# Autodesk Inventor assembly: Trunk
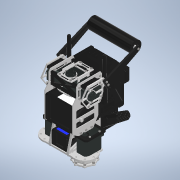
[picture p0: Inventor's stored thumbnail of the model, 180x180]
Saved by Autodesk Inventor 2020.4 (Build 244396000, 396)
## iProperties
Created: 2021-09-10
Part Number: Trunk
Document SubType Name: Assembly
Designer: Masato
Mass: 1663.74 g
Surface Area: 5902.56 cm^2
Volume: 962.647 cm^3
Density: 1.72829 g/cm^3
Author: Masato
## Documents named in this file (38)
- C:\Users\Masato\Documents\Inventor\CIT Brains_Inventor\OpenPlatform_ver3_0\UpperBody\Trunk\Trunk.iam
- C:\Users\Masato\Documents\Inventor\CIT Brains_Inventor\OpenPlatform_ver3_0\UpperBody\Trunk\Trunk_horizontal_frame_02.ipt
- C:\Users\Masato\Documents\Inventor\CIT Brains_Inventor\OpenPlatform_ver3_0\UpperBody\Trunk\Trunk_horizontal_frame_03.ipt
- C:\Users\Masato\Documents\Inventor\CIT Brains_Inventor\OpenPlatform_ver3_0\UpperBody\Trunk\Trunk_horizontal_frame_04.ipt
- C:\Users\Masato\Documents\Inventor\CIT Brains_Inventor\OpenPlatform_ver3_0\UpperBody\Trunk\Trunk_horizontal_frame_05.ipt
- C:\Users\Masato\Documents\Inventor\CIT Brains_Inventor\OpenPlatform_ver3_0\UpperBody\Trunk\Trunk_vertical_frame_02.ipt
- C:\Users\Masato\Documents\Inventor\CIT Brains_Inventor\OpenPlatform_ver3_0\UpperBody\Trunk\Trunk_vertical_frame_03.ipt
- C:\Users\Masato\Documents\Inventor\CIT Brains_Inventor\OpenPlatform_ver3_0\UpperBody\Trunk\Trunk_vertical_frame_04.ipt
- C:\Users\Masato\Documents\Inventor\CIT Brains_Inventor\OpenPlatform_ver3_0\UpperBody\Trunk\Trunk_vertical_frame_05.ipt
- C:\Users\Masato\Documents\Inventor\CIT Brains_Inventor\OpenPlatform_ver3_0\UpperBody\Trunk\Trunk_vertical_frame_06.ipt
- C:\Users\Masato\Documents\Inventor\CIT Brains_Inventor\OpenPlatform_ver3_0\Ready_Made\B3M11xx.ipt
- C:\Users\Masato\Documents\Inventor\CIT Brains_Inventor\OpenPlatform_ver3_0\Ready_Made\S3-07-3W.ipt
- C:\Users\Masato\Documents\Inventor\CIT Brains_Inventor\OpenPlatform_ver3_0\Ready_Made\ASU-375H.ipt
- C:\Users\Masato\Documents\Inventor\CIT Brains_Inventor\OpenPlatform_ver3_0\UpperBody\Trunk\RearBumper.ipt
- C:\Users\Masato\Documents\Inventor\CIT Brains_Inventor\OpenPlatform_ver3_0\UpperBody\Trunk\RearBumper_MIR.ipt
- C:\Users\Masato\Documents\Inventor\CIT Brains_Inventor\OpenPlatform_ver3_0\Ready_Made\MSU-306-03.ipt
- C:\Users\Masato\Documents\Inventor\CIT Brains_Inventor\OpenPlatform_ver3_0\Ready_Made\SLSBF7-130-M3-N3.ipt
- C:\Users\Masato\Documents\Inventor\CIT Brains_Inventor\OpenPlatform_ver3_0\Ready_Made\B3M10xx.ipt
- C:\Users\Masato\Documents\Inventor\CIT Brains_Inventor\OpenPlatform_ver3_0\Ready_Made\SGB-100.ipt
- C:\Users\Masato\Documents\Inventor\CIT Brains_Inventor\OpenPlatform_ver3_0\UpperBody\Cockpit\Cockpit.iam
- C:\Users\Masato\Documents\Inventor\CIT Brains_Inventor\OpenPlatform_ver3_0\UpperBody\Trunk\Trunk_vertical_frame_04_MIR.ipt
- C:\Users\Masato\Documents\Inventor\CIT Brains_Inventor\OpenPlatform_ver3_0\UpperBody\Trunk\Trunk_vertical_frame_01.ipt
- C:\Users\Masato\Documents\Inventor\CIT Brains_Inventor\OpenPlatform_ver3_0\UpperBody\Trunk\Trunk_vertical_frame_01_MIR.ipt
- C:\Users\Masato\Documents\Inventor\CIT Brains_Inventor\OpenPlatform_ver3_0\Ready_Made\Screw\SPNFL-BRN-M3-6.ipt
- C:\Users\Masato\Documents\Inventor\CIT Brains_Inventor\OpenPlatform_ver3_0\Ready_Made\Screw\M2_6-15.ipt
- C:\Users\Masato\Documents\Inventor\CIT Brains_Inventor\OpenPlatform_ver3_0\Ready_Made\Screw\M3-8.ipt
- C:\Users\Masato\Documents\Inventor\CIT Brains_Inventor\OpenPlatform_ver3_0\Ready_Made\Screw\M3-6.ipt
- C:\Users\Masato\Documents\Inventor\CIT Brains_Inventor\OpenPlatform_ver3_0\Ready_Made\Screw\M2_6-20.ipt
- C:\Users\Masato\Documents\Inventor\CIT Brains_Inventor\OpenPlatform_ver3_0\UpperBody\Trunk\Outer_support_stand.ipt
- C:\Users\Masato\Documents\Inventor\CIT Brains_Inventor\OpenPlatform_ver3_0\Ready_Made\BRU-307S.ipt
- C:\Users\Masato\Documents\Inventor\CIT Brains_Inventor\OpenPlatform_ver3_0\UpperBody\Trunk\Outer_flange.ipt
- C:\Users\Masato\Documents\Inventor\CIT Brains_Inventor\OpenPlatform_ver3_0\UpperBody\Trunk\Inner_flange.ipt
- C:\Users\Masato\Documents\Inventor\CIT Brains_Inventor\OpenPlatform_ver3_0\Ready_Made\CRBA02508WWC8P5\CRBA02508WWC8P5.ipt
- C:\Users\Masato\Documents\Inventor\CIT Brains_Inventor\OpenPlatform_ver3_0\UpperBody\Trunk\Inner_support_stand.ipt
- C:\Users\Masato\Documents\Inventor\CIT Brains_Inventor\OpenPlatform_ver3_0\UpperBody\Trunk\Trunk_horizontal_frame_01.ipt
- C:\Users\Masato\Documents\Inventor\CIT Brains_Inventor\OpenPlatform_ver3_0\Ready_Made\SF319.ipt
- C:\Users\Masato\Documents\Inventor\CIT Brains_Inventor\OpenPlatform_ver3_0\Ready_Made\BRU-2609S.ipt
- C:\Users\Masato\Documents\Inventor\CIT Brains_Inventor\OpenPlatform_ver3_0\Ready_Made\Screw\M2_6-8.ipt
## Components (174 placed, 37 different names)
1. Trunk_horizontal_frame_02:1 — 挿入:9, 挿入:10, 挿入:11, 挿入:12, 挿入:269, 挿入:270, 挿入:271, 挿入:272
2. Trunk_horizontal_frame_03:1 — 挿入:172, 挿入:173, 挿入:174, 挿入:175, 挿入:176, 挿入:177, 挿入:178, 挿入:179, 挿入:255, 挿入:256, 挿入:259, 挿入:260, 挿入:261, 挿入:262, 挿入:347, 挿入:348
3. Trunk_horizontal_frame_03:2 — 挿入:180, 挿入:181, 挿入:182, 挿入:183, 挿入:184, 挿入:185, 挿入:186, 挿入:187, 挿入:257, 挿入:258, 挿入:335, 挿入:336, 挿入:337, 挿入:338
4. Trunk_horizontal_frame_04:1 — 挿入:115, 挿入:116, 挿入:117, 挿入:118, 挿入:172, 挿入:173, 挿入:181, 挿入:182
5. Trunk_horizontal_frame_04:2 — 挿入:154, 挿入:155, 挿入:156, 挿入:157, 挿入:174, 挿入:175, 挿入:185, 挿入:187
6. Trunk_horizontal_frame_05:1 — 挿入:111, 挿入:112, 挿入:126, 挿入:127
7. Trunk_horizontal_frame_05:2 — 挿入:162, 挿入:163, 挿入:164, 挿入:165
8. Trunk_horizontal_frame_05:3 — 挿入:229, 挿入:230, 挿入:231, 挿入:232
9. Trunk_horizontal_frame_05:4 — 挿入:166, 挿入:167, 挿入:168, 挿入:169
10. Trunk_vertical_frame_01:1 — 角度:35, 角度:36, 挿入:200, 挿入:201, 挿入:206, 挿入:207, 挿入:420, 挿入:421, 挿入:426
11. Trunk_vertical_frame_01_MIR:1 — 角度:37, 角度:38, 挿入:202, 挿入:203, 挿入:204, 挿入:205, メイト:23, メイト:24, メイト:25, 挿入:418, 挿入:419
12. Trunk_vertical_frame_02:1 — フラッシュ:16, メイト:17, フラッシュ:18, フラッシュ:20, フラッシュ:21, メイト:22
13. Trunk_vertical_frame_02:2 — フラッシュ:16, メイト:17, フラッシュ:18, メイト:19
14. Trunk_vertical_frame_02:3 — フラッシュ:15, メイト:18, フラッシュ:17, フラッシュ:19, フラッシュ:20, フラッシュ:21, メイト:21, メイト:20
15. Trunk_vertical_frame_02:4 — フラッシュ:15, メイト:18, フラッシュ:17, メイト:25
16. Trunk_vertical_frame_03:1 — 挿入:101, 挿入:102, 挿入:103, 挿入:111, 挿入:112, 挿入:115, 挿入:116, 挿入:156, 挿入:157, 挿入:164, 挿入:165, フラッシュ:19, メイト:21, 挿入:208, 挿入:226, 挿入:245, 挿入:246, 挿入:247, 挿入:251, 挿入:252, 挿入:327, 挿入:328, 挿入:329, 挿入:330, 挿入:349, 挿入:350
17. Trunk_vertical_frame_03:2 — 挿入:104, 挿入:105, 挿入:106, 挿入:117, 挿入:118, 挿入:154, 挿入:155, 挿入:168, 挿入:169, メイト:22, 挿入:227, 挿入:229, 挿入:230, 挿入:248, 挿入:249, 挿入:250, 挿入:253, 挿入:254, 挿入:331, 挿入:332, 挿入:333, 挿入:334, 挿入:351, 挿入:352
18. Trunk_vertical_frame_04:1 — 挿入:142, 挿入:143, 挿入:144, 挿入:145, 角度:31, 角度:32, 挿入:150, 挿入:151, 挿入:166, 挿入:167, 挿入:231, 挿入:232, 挿入:315, 挿入:316, 挿入:317, 挿入:318, 挿入:323, 挿入:324, 挿入:325, 挿入:326
19. Trunk_vertical_frame_04_MIR:1 — 挿入:124, 挿入:125, 挿入:126, 挿入:127, 挿入:128, 挿入:129, 挿入:136, 挿入:137, 角度:33, 角度:34, 挿入:152, 挿入:153, 挿入:162, 挿入:163, 挿入:311, 挿入:312, 挿入:313, 挿入:314, 挿入:319, 挿入:320, 挿入:321, 挿入:322
20. Trunk_vertical_frame_05:1 — 角度:17, 角度:18, 挿入:75, 挿入:76, 角度:21, 挿入:79, メイト:16, 挿入:263, 挿入:264, 挿入:267
21. Trunk_vertical_frame_05:2 — 角度:19, 挿入:77, 挿入:78, 角度:20, 角度:22, 挿入:80, 挿入:265, 挿入:266, 挿入:268
22. Trunk_vertical_frame_06:1 — 挿入:192, 挿入:193, 挿入:194, 挿入:195, 挿入:343, 挿入:344, 挿入:345, 挿入:346
23. Trunk_vertical_frame_06:2 — 挿入:188, 挿入:189, 挿入:190, 挿入:191, 挿入:339, 挿入:340, 挿入:341, 挿入:342
24. RearBumper:1 — 挿入:204, 挿入:205
25. RearBumper_MIR:1 — 挿入:206, 挿入:207
26. B3M11xx:1 — 挿入:11, 挿入:12, 角度:39, 挿入:391, 挿入:392, 挿入:422, 挿入:423, 挿入:424, 挿入:425
27. B3M11xx:2 — 挿入:9, 挿入:10, 挿入:427, 挿入:428, 挿入:429
28. B3M11xx:3 — 挿入:176, 挿入:177, 挿入:178, 挿入:179, 挿入:180, 挿入:183, 挿入:184, 挿入:186
29. B3M10xx:4 — 挿入:124, 挿入:125, 挿入:128, 挿入:129, 挿入:188, 挿入:189, 挿入:190, 挿入:191
30. B3M10xx:5 — 挿入:142, 挿入:143, 挿入:144, 挿入:145, 挿入:192, 挿入:193, 挿入:194, 挿入:195
31. S3-07-3W:1 — 角度:37, 挿入:202
32. S3-07-3W:2 — 角度:38, 挿入:203
33. S3-07-3W:3 — 角度:36, 挿入:201
34. S3-07-3W:4 — 角度:35, 挿入:200
35. S3-07-3W:5 — 角度:33, 挿入:152
36. S3-07-3W:6 — 角度:34, 挿入:153
37. S3-07-3W:7 — 角度:31, 挿入:150
38. S3-07-3W:8 — 角度:32, 挿入:151
39. ASU-375H:1 — フラッシュ:9, フラッシュ:10, フラッシュ:11, フラッシュ:12, 挿入:101, 挿入:104, メイト:19, メイト:20, メイト:23, メイト:24
40. ASU-375H:2 — フラッシュ:9, フラッシュ:11, 挿入:102, 挿入:105
41. ASU-375H:3 — フラッシュ:10, フラッシュ:12, 挿入:103, 挿入:106
42. MSU-306-03:5 — 角度:17, 挿入:75, 挿入:136
43. MSU-306-03:6 — 角度:18, 挿入:76, 挿入:137
44. MSU-306-03:11 — 角度:19, 挿入:77
45. MSU-306-03:12 — 挿入:78, 角度:20
46. SLSBF7-130-M3-N3:1 — 角度:21, 角度:22, 挿入:79, 挿入:80, メイト:15
47. SGB-100:1 — メイト:15, メイト:16
48. Cockpit:1 [sub-assembly] — 挿入:208, 角度:39
49. SPNFL-BRN-M3-6:1 — 挿入:226
50. SPNFL-BRN-M3-6:2 — 挿入:227
51. M3-8:5 — 挿入:245
52. M3-8:6 — 挿入:246
53. M3-8:7 — 挿入:247
54. M3-8:8 — 挿入:248
55. M3-8:9 — 挿入:249
56. M3-8:10 — 挿入:250
57. M3-6:1 — 挿入:251
58. M3-6:2 — 挿入:252
59. M3-6:3 — 挿入:254
60. M3-6:4 — 挿入:253
61. M3-6:5 — 挿入:256
62. M3-6:6 — 挿入:255
63. M3-6:7 — 挿入:258
64. M3-6:8 — 挿入:257
65. M2_6-15:9 — 挿入:259
66. M2_6-15:10 — 挿入:260
67. M2_6-15:11 — 挿入:261
68. M2_6-15:12 — 挿入:262
69. M3-6:9 — 挿入:263
70. M3-6:10 — 挿入:264
71. M3-6:11 — 挿入:266
72. M3-6:12 — 挿入:265
73. M3-8:11 — 挿入:267
74. M3-8:12 — 挿入:268
75. M2_6-20:1 — 挿入:269
76. M2_6-20:2 — 挿入:270
77. M2_6-20:3 — 挿入:272
78. M2_6-20:4 — 挿入:271
79. M2_6-15:13 — 挿入:311
80. M2_6-15:14 — 挿入:312
81. M2_6-15:15 — 挿入:313
82. M2_6-15:16 — 挿入:314
83. M2_6-15:17 — 挿入:315
84. M2_6-15:18 — 挿入:316
85. M2_6-15:19 — 挿入:317
86. M2_6-15:20 — 挿入:318
87. M3-6:13 — 挿入:319
88. M3-6:14 — 挿入:320
89. M3-6:15 — 挿入:321
90. M3-6:16 — 挿入:322
91. M3-6:17 — 挿入:323
92. M3-6:18 — 挿入:324
93. M3-6:19 — 挿入:325
94. M3-6:20 — 挿入:326
95. M3-6:21 — 挿入:327
96. M3-6:22 — 挿入:328
97. M3-6:23 — 挿入:329
98. M3-6:24 — 挿入:330
99. M3-6:25 — 挿入:331
100. M3-6:26 — 挿入:332
101. M3-6:27 — 挿入:333
102. M3-6:28 — 挿入:334
103. M2_6-20:9 — 挿入:335
104. M2_6-20:10 — 挿入:336
105. M2_6-20:11 — 挿入:337
106. M2_6-20:12 — 挿入:338
107. M2_6-20:13 — 挿入:339
108. M2_6-20:14 — 挿入:342
109. M2_6-20:15 — 挿入:341
110. M2_6-20:16 — 挿入:340
111. M2_6-20:17 — 挿入:344
112. M2_6-20:18 — 挿入:345
113. M2_6-20:19 — 挿入:346
114. M2_6-20:20 — 挿入:343
115. M3-6:29 — 挿入:347
116. M3-6:30 — 挿入:348
117. M3-6:31 — 挿入:349
118. M3-6:32 — 挿入:350
119. M3-6:33 — 挿入:351
120. M3-6:34 — 挿入:352
121. Outer_support_stand:1 — 挿入:371, 挿入:372, 挿入:373, 挿入:374, 挿入:375, 挿入:376, 挿入:377, 挿入:378, 挿入:397, 挿入:438, 挿入:439
122. BRU-307S:1 — 挿入:371, 挿入:404
123. BRU-307S:2 — 挿入:372
124. BRU-307S:3 — 挿入:373
125. BRU-307S:4 — 挿入:374
126. BRU-307S:5 — 挿入:375, 挿入:405
127. BRU-307S:6 — 挿入:376
128. BRU-307S:7 — 挿入:377
129. BRU-307S:8 — 挿入:378
130. Inner_flange:1 — 挿入:391, 挿入:392, 挿入:452, 挿入:453, 挿入:454, 挿入:455
131. CRBA02508WWC8P5:1 — 挿入:397
132. Inner_support_stand:1 — 角度:40, 挿入:398, 角度:41, 挿入:399, 角度:42, 挿入:400, 角度:43, 挿入:401, 挿入:456, 挿入:457, 挿入:458, 挿入:459, 挿入:460, 挿入:461
133. S3-07-3W:9 — 角度:40, 挿入:398
134. S3-07-3W:10 — 角度:41, 挿入:399
135. S3-07-3W:11 — 角度:42, 挿入:400
136. S3-07-3W:12 — 角度:43, 挿入:401
137. Outer_flange:1 — 挿入:404, 挿入:405, 挿入:406, 挿入:407, 挿入:408, 挿入:409, 挿入:410, 挿入:411, 挿入:412, 挿入:413
138. M3-6:35 — 挿入:406
139. M3-6:36 — 挿入:407
140. M3-6:37 — 挿入:408
141. M3-6:38 — 挿入:409
142. M3-6:39 — 挿入:410
143. M3-6:40 — 挿入:411
144. M3-6:41 — 挿入:412
145. M3-6:42 — 挿入:413
146. Trunk_horizontal_frame_01:1 — 挿入:418, 挿入:419, 挿入:420, 挿入:421, 挿入:422, 挿入:423, 挿入:424, 挿入:425, 挿入:426, 挿入:427, 挿入:428, 挿入:429, 挿入:430, 挿入:431, 挿入:432, 挿入:433, 挿入:434, 挿入:435, 挿入:436, 挿入:440, 挿入:441, 挿入:442, 挿入:443, 挿入:444, 挿入:445, 挿入:446, 挿入:447, 挿入:448, 挿入:449, 挿入:450, 挿入:451, フラッシュ:22, 挿入:462
147. SF319:1 — 挿入:430
148. SF319:2 — 挿入:431
149. SF319:3 — 挿入:432
150. SF319:4 — 挿入:433, 挿入:439
151. SF319:5 — 挿入:434
152. SF319:6 — 挿入:435
153. SF319:7 — 挿入:436, 挿入:438
154. SF319:8 — 挿入:462
155. M2_6-15:21 — 挿入:441
156. M2_6-15:22 — 挿入:440
157. M2_6-15:23 — 挿入:442
158. M2_6-15:24 — 挿入:443
159. M2_6-15:25 — 挿入:444
160. M2_6-15:26 — 挿入:445
161. M2_6-15:27 — 挿入:446
162. M2_6-15:28 — 挿入:447
163. M3-8:13 — 挿入:448
164. M3-8:14 — 挿入:449
165. M3-8:15 — 挿入:450
166. M3-8:16 — 挿入:451
167. BRU-2609S:1 — 挿入:455, 挿入:457
168. BRU-2609S:2 — 挿入:454
169. BRU-2609S:3 — 挿入:453
170. BRU-2609S:4 — 挿入:452, 挿入:456
171. M2_6-8:1 — 挿入:458
172. M2_6-8:2 — 挿入:459
173. M2_6-8:3 — 挿入:460
174. M2_6-8:4 — 挿入:461
## Relationships (270: Insert 228, Angle 19, Flush 12, Mate 11)
- 挿入:9 [Insert]: Trunk_horizontal_frame_02:1 ↔ B3M11xx:2
- 挿入:10 [Insert]: Trunk_horizontal_frame_02:1 ↔ B3M11xx:2
- 挿入:11 [Insert]: Trunk_horizontal_frame_02:1 ↔ B3M11xx:1
- 挿入:12 [Insert]: Trunk_horizontal_frame_02:1 ↔ B3M11xx:1
- フラッシュ:9 [Flush]: ASU-375H:1 ↔ ASU-375H:2
- フラッシュ:10 [Flush]: ASU-375H:1 ↔ ASU-375H:3
- フラッシュ:11 [Flush]: ASU-375H:1 ↔ ASU-375H:2
- フラッシュ:12 [Flush]: ASU-375H:1 ↔ ASU-375H:3
- 角度:17 [Angle] (0 deg): Trunk_vertical_frame_05:1 ↔ MSU-306-03:5
- 角度:18 [Angle] (0 deg): Trunk_vertical_frame_05:1 ↔ MSU-306-03:6
- 挿入:75 [Insert]: Trunk_vertical_frame_05:1 ↔ MSU-306-03:5
- 挿入:76 [Insert]: Trunk_vertical_frame_05:1 ↔ MSU-306-03:6
- 角度:19 [Angle] (0 deg): Trunk_vertical_frame_05:2 ↔ MSU-306-03:11
- 挿入:77 [Insert]: Trunk_vertical_frame_05:2 ↔ MSU-306-03:11
- 挿入:78 [Insert]: Trunk_vertical_frame_05:2 ↔ MSU-306-03:12
- 角度:20 [Angle] (0 deg): Trunk_vertical_frame_05:2 ↔ MSU-306-03:12
- 角度:21 [Angle] (0 deg): Trunk_vertical_frame_05:1 ↔ SLSBF7-130-M3-N3:1
- 角度:22 [Angle] (0 deg): Trunk_vertical_frame_05:2 ↔ SLSBF7-130-M3-N3:1
- 挿入:79 [Insert]: Trunk_vertical_frame_05:1 ↔ SLSBF7-130-M3-N3:1
- 挿入:80 [Insert]: Trunk_vertical_frame_05:2 ↔ SLSBF7-130-M3-N3:1
- メイト:15 [Mate]: SLSBF7-130-M3-N3:1 ↔ SGB-100:1
- メイト:16 [Mate] (2.5 mm): Trunk_vertical_frame_05:1 ↔ SGB-100:1
- 挿入:101 [Insert]: Trunk_vertical_frame_03:1 ↔ ASU-375H:1
- 挿入:102 [Insert]: Trunk_vertical_frame_03:1 ↔ ASU-375H:2
- 挿入:103 [Insert]: Trunk_vertical_frame_03:1 ↔ ASU-375H:3
- 挿入:104 [Insert]: Trunk_vertical_frame_03:2 ↔ ASU-375H:1
- 挿入:105 [Insert]: Trunk_vertical_frame_03:2 ↔ ASU-375H:2
- 挿入:106 [Insert]: Trunk_vertical_frame_03:2 ↔ ASU-375H:3
- 挿入:111 [Insert]: Trunk_horizontal_frame_05:1 ↔ Trunk_vertical_frame_03:1
- 挿入:112 [Insert]: Trunk_horizontal_frame_05:1 ↔ Trunk_vertical_frame_03:1
- 挿入:115 [Insert]: Trunk_horizontal_frame_04:1 ↔ Trunk_vertical_frame_03:1
- 挿入:116 [Insert]: Trunk_horizontal_frame_04:1 ↔ Trunk_vertical_frame_03:1
- 挿入:117 [Insert]: Trunk_horizontal_frame_04:1 ↔ Trunk_vertical_frame_03:2
- 挿入:118 [Insert]: Trunk_horizontal_frame_04:1 ↔ Trunk_vertical_frame_03:2
- 挿入:124 [Insert]: Trunk_vertical_frame_04_MIR:1 ↔ B3M10xx:4
- 挿入:125 [Insert]: Trunk_vertical_frame_04_MIR:1 ↔ B3M10xx:4
- 挿入:126 [Insert]: Trunk_horizontal_frame_05:1 ↔ Trunk_vertical_frame_04_MIR:1
- 挿入:127 [Insert]: Trunk_horizontal_frame_05:1 ↔ Trunk_vertical_frame_04_MIR:1
- 挿入:128 [Insert]: Trunk_vertical_frame_04_MIR:1 ↔ B3M10xx:4
- 挿入:129 [Insert]: Trunk_vertical_frame_04_MIR:1 ↔ B3M10xx:4
- 挿入:136 [Insert]: Trunk_vertical_frame_04_MIR:1 ↔ MSU-306-03:5
- 挿入:137 [Insert]: Trunk_vertical_frame_04_MIR:1 ↔ MSU-306-03:6
- 挿入:142 [Insert]: Trunk_vertical_frame_04:1 ↔ B3M10xx:5
- 挿入:143 [Insert]: Trunk_vertical_frame_04:1 ↔ B3M10xx:5
- 挿入:144 [Insert]: Trunk_vertical_frame_04:1 ↔ B3M10xx:5
- 挿入:145 [Insert]: Trunk_vertical_frame_04:1 ↔ B3M10xx:5
- 角度:31 [Angle] (0 deg): Trunk_vertical_frame_04:1 ↔ S3-07-3W:7
- 角度:32 [Angle] (0 deg): Trunk_vertical_frame_04:1 ↔ S3-07-3W:8
- 挿入:150 [Insert]: Trunk_vertical_frame_04:1 ↔ S3-07-3W:7
- 挿入:151 [Insert]: Trunk_vertical_frame_04:1 ↔ S3-07-3W:8
- 角度:33 [Angle] (0 deg): Trunk_vertical_frame_04_MIR:1 ↔ S3-07-3W:5
- 角度:34 [Angle] (0 deg): Trunk_vertical_frame_04_MIR:1 ↔ S3-07-3W:6
- 挿入:152 [Insert]: Trunk_vertical_frame_04_MIR:1 ↔ S3-07-3W:5
- 挿入:153 [Insert]: Trunk_vertical_frame_04_MIR:1 ↔ S3-07-3W:6
- 挿入:154 [Insert]: Trunk_horizontal_frame_04:2 ↔ Trunk_vertical_frame_03:2
- 挿入:155 [Insert]: Trunk_horizontal_frame_04:2 ↔ Trunk_vertical_frame_03:2
- 挿入:156 [Insert]: Trunk_horizontal_frame_04:2 ↔ Trunk_vertical_frame_03:1
- 挿入:157 [Insert]: Trunk_horizontal_frame_04:2 ↔ Trunk_vertical_frame_03:1
- 挿入:162 [Insert]: Trunk_horizontal_frame_05:2 ↔ Trunk_vertical_frame_04_MIR:1
- 挿入:163 [Insert]: Trunk_horizontal_frame_05:2 ↔ Trunk_vertical_frame_04_MIR:1
- 挿入:164 [Insert]: Trunk_horizontal_frame_05:2 ↔ Trunk_vertical_frame_03:1
- 挿入:165 [Insert]: Trunk_horizontal_frame_05:2 ↔ Trunk_vertical_frame_03:1
- 挿入:166 [Insert]: Trunk_horizontal_frame_05:4 ↔ Trunk_vertical_frame_04:1
- 挿入:167 [Insert]: Trunk_horizontal_frame_05:4 ↔ Trunk_vertical_frame_04:1
- 挿入:168 [Insert]: Trunk_horizontal_frame_05:4 ↔ Trunk_vertical_frame_03:2
- 挿入:169 [Insert]: Trunk_horizontal_frame_05:4 ↔ Trunk_vertical_frame_03:2
- 挿入:172 [Insert]: Trunk_horizontal_frame_03:1 ↔ Trunk_horizontal_frame_04:1
- 挿入:173 [Insert]: Trunk_horizontal_frame_03:1 ↔ Trunk_horizontal_frame_04:1
- 挿入:174 [Insert]: Trunk_horizontal_frame_03:1 ↔ Trunk_horizontal_frame_04:2
- 挿入:175 [Insert]: Trunk_horizontal_frame_03:1 ↔ Trunk_horizontal_frame_04:2
- 挿入:176 [Insert]: Trunk_horizontal_frame_03:1 ↔ B3M11xx:3
- 挿入:177 [Insert]: Trunk_horizontal_frame_03:1 ↔ B3M11xx:3
- 挿入:178 [Insert]: Trunk_horizontal_frame_03:1 ↔ B3M11xx:3
- 挿入:179 [Insert]: Trunk_horizontal_frame_03:1 ↔ B3M11xx:3
- 挿入:180 [Insert]: Trunk_horizontal_frame_03:2 ↔ B3M11xx:3
- 挿入:181 [Insert]: Trunk_horizontal_frame_03:2 ↔ Trunk_horizontal_frame_04:1
- 挿入:182 [Insert]: Trunk_horizontal_frame_03:2 ↔ Trunk_horizontal_frame_04:1
- 挿入:183 [Insert]: Trunk_horizontal_frame_03:2 ↔ B3M11xx:3
- 挿入:184 [Insert]: Trunk_horizontal_frame_03:2 ↔ B3M11xx:3
- 挿入:185 [Insert]: Trunk_horizontal_frame_03:2 ↔ Trunk_horizontal_frame_04:2
- 挿入:186 [Insert]: Trunk_horizontal_frame_03:2 ↔ B3M11xx:3
- 挿入:187 [Insert]: Trunk_horizontal_frame_03:2 ↔ Trunk_horizontal_frame_04:2
- 挿入:188 [Insert]: Trunk_vertical_frame_06:2 ↔ B3M10xx:4
- 挿入:189 [Insert]: Trunk_vertical_frame_06:2 ↔ B3M10xx:4
- 挿入:190 [Insert]: Trunk_vertical_frame_06:2 ↔ B3M10xx:4
- 挿入:191 [Insert]: Trunk_vertical_frame_06:2 ↔ B3M10xx:4
- 挿入:192 [Insert]: Trunk_vertical_frame_06:1 ↔ B3M10xx:5
- 挿入:193 [Insert]: Trunk_vertical_frame_06:1 ↔ B3M10xx:5
- 挿入:194 [Insert]: Trunk_vertical_frame_06:1 ↔ B3M10xx:5
- 挿入:195 [Insert]: Trunk_vertical_frame_06:1 ↔ B3M10xx:5
- フラッシュ:15 [Flush]: Trunk_vertical_frame_02:3 ↔ Trunk_vertical_frame_02:4
- フラッシュ:16 [Flush]: Trunk_vertical_frame_02:1 ↔ Trunk_vertical_frame_02:2
- メイト:17 [Mate]: Trunk_vertical_frame_02:1 ↔ Trunk_vertical_frame_02:2
- メイト:18 [Mate]: Trunk_vertical_frame_02:3 ↔ Trunk_vertical_frame_02:4
- フラッシュ:17 [Flush]: Trunk_vertical_frame_02:3 ↔ Trunk_vertical_frame_02:4
- フラッシュ:18 [Flush]: Trunk_vertical_frame_02:1 ↔ Trunk_vertical_frame_02:2
- フラッシュ:19 [Flush]: Trunk_vertical_frame_02:3 ↔ Trunk_vertical_frame_03:1
- フラッシュ:20 [Flush]: Trunk_vertical_frame_02:1 ↔ Trunk_vertical_frame_02:3
- メイト:19 [Mate] (0.01 mm): Trunk_vertical_frame_02:2 ↔ ASU-375H:1
- メイト:20 [Mate] (0.01 mm): Trunk_vertical_frame_02:3 ↔ ASU-375H:1
- フラッシュ:21 [Flush]: Trunk_vertical_frame_02:1 ↔ Trunk_vertical_frame_02:3
- メイト:21 [Mate]: Trunk_vertical_frame_02:3 ↔ Trunk_vertical_frame_03:1
- メイト:22 [Mate]: Trunk_vertical_frame_02:1 ↔ Trunk_vertical_frame_03:2
- 角度:35 [Angle] (0 deg): Trunk_vertical_frame_01:1 ↔ S3-07-3W:4
- 角度:36 [Angle] (0 deg): Trunk_vertical_frame_01:1 ↔ S3-07-3W:3
- 挿入:200 [Insert]: Trunk_vertical_frame_01:1 ↔ S3-07-3W:4
- 挿入:201 [Insert]: Trunk_vertical_frame_01:1 ↔ S3-07-3W:3
- 角度:37 [Angle] (0 deg): Trunk_vertical_frame_01_MIR:1 ↔ S3-07-3W:1
- 角度:38 [Angle] (0 deg): Trunk_vertical_frame_01_MIR:1 ↔ S3-07-3W:2
- 挿入:202 [Insert]: Trunk_vertical_frame_01_MIR:1 ↔ S3-07-3W:1
- 挿入:203 [Insert]: Trunk_vertical_frame_01_MIR:1 ↔ S3-07-3W:2
- 挿入:204 [Insert]: Trunk_vertical_frame_01_MIR:1 ↔ RearBumper:1
- 挿入:205 [Insert]: Trunk_vertical_frame_01_MIR:1 ↔ RearBumper:1
- 挿入:206 [Insert]: Trunk_vertical_frame_01:1 ↔ RearBumper_MIR:1
- 挿入:207 [Insert]: Trunk_vertical_frame_01:1 ↔ RearBumper_MIR:1
- メイト:23 [Mate] (0.01 mm): Trunk_vertical_frame_01_MIR:1 ↔ ASU-375H:1
- メイト:24 [Mate] (0.01 mm): Trunk_vertical_frame_01_MIR:1 ↔ ASU-375H:1
- メイト:25 [Mate]: Trunk_vertical_frame_01_MIR:1 ↔ Trunk_vertical_frame_02:4
- 挿入:208 [Insert] (0.25 mm): Trunk_vertical_frame_03:1 ↔ Cockpit:1
- 角度:39 [Angle] (0 deg): B3M11xx:1 ↔ Cockpit:1
- 挿入:226 [Insert]: Trunk_vertical_frame_03:1 ↔ SPNFL-BRN-M3-6:1
- 挿入:227 [Insert]: Trunk_vertical_frame_03:2 ↔ SPNFL-BRN-M3-6:2
- 挿入:229 [Insert]: Trunk_horizontal_frame_05:3 ↔ Trunk_vertical_frame_03:2
- 挿入:230 [Insert]: Trunk_horizontal_frame_05:3 ↔ Trunk_vertical_frame_03:2
- 挿入:231 [Insert]: Trunk_horizontal_frame_05:3 ↔ Trunk_vertical_frame_04:1
- 挿入:232 [Insert]: Trunk_horizontal_frame_05:3 ↔ Trunk_vertical_frame_04:1
- 挿入:245 [Insert]: Trunk_vertical_frame_03:1 ↔ M3-8:5
- 挿入:246 [Insert]: Trunk_vertical_frame_03:1 ↔ M3-8:6
- 挿入:247 [Insert]: Trunk_vertical_frame_03:1 ↔ M3-8:7
- 挿入:248 [Insert]: Trunk_vertical_frame_03:2 ↔ M3-8:8
- 挿入:249 [Insert]: Trunk_vertical_frame_03:2 ↔ M3-8:9
- 挿入:250 [Insert]: Trunk_vertical_frame_03:2 ↔ M3-8:10
- 挿入:251 [Insert]: Trunk_vertical_frame_03:1 ↔ M3-6:1
- 挿入:252 [Insert]: Trunk_vertical_frame_03:1 ↔ M3-6:2
- 挿入:253 [Insert]: Trunk_vertical_frame_03:2 ↔ M3-6:4
- 挿入:254 [Insert]: Trunk_vertical_frame_03:2 ↔ M3-6:3
- 挿入:255 [Insert]: Trunk_horizontal_frame_03:1 ↔ M3-6:6
- 挿入:256 [Insert]: Trunk_horizontal_frame_03:1 ↔ M3-6:5
- 挿入:257 [Insert]: Trunk_horizontal_frame_03:2 ↔ M3-6:8
- 挿入:258 [Insert]: Trunk_horizontal_frame_03:2 ↔ M3-6:7
- 挿入:259 [Insert]: Trunk_horizontal_frame_03:1 ↔ M2_6-15:9
- 挿入:260 [Insert]: Trunk_horizontal_frame_03:1 ↔ M2_6-15:10
- 挿入:261 [Insert]: Trunk_horizontal_frame_03:1 ↔ M2_6-15:11
- 挿入:262 [Insert]: Trunk_horizontal_frame_03:1 ↔ M2_6-15:12
- 挿入:263 [Insert]: Trunk_vertical_frame_05:1 ↔ M3-6:9
- 挿入:264 [Insert]: Trunk_vertical_frame_05:1 ↔ M3-6:10
- 挿入:265 [Insert]: Trunk_vertical_frame_05:2 ↔ M3-6:12
- 挿入:266 [Insert]: Trunk_vertical_frame_05:2 ↔ M3-6:11
- 挿入:267 [Insert]: Trunk_vertical_frame_05:1 ↔ M3-8:11
- 挿入:268 [Insert]: Trunk_vertical_frame_05:2 ↔ M3-8:12
- 挿入:269 [Insert]: Trunk_horizontal_frame_02:1 ↔ M2_6-20:1
- 挿入:270 [Insert]: Trunk_horizontal_frame_02:1 ↔ M2_6-20:2
- 挿入:271 [Insert]: Trunk_horizontal_frame_02:1 ↔ M2_6-20:4
- 挿入:272 [Insert]: Trunk_horizontal_frame_02:1 ↔ M2_6-20:3
- 挿入:311 [Insert]: Trunk_vertical_frame_04_MIR:1 ↔ M2_6-15:13
- 挿入:312 [Insert]: Trunk_vertical_frame_04_MIR:1 ↔ M2_6-15:14
- 挿入:313 [Insert]: Trunk_vertical_frame_04_MIR:1 ↔ M2_6-15:15
- 挿入:314 [Insert]: Trunk_vertical_frame_04_MIR:1 ↔ M2_6-15:16
- 挿入:315 [Insert]: Trunk_vertical_frame_04:1 ↔ M2_6-15:17
- 挿入:316 [Insert]: Trunk_vertical_frame_04:1 ↔ M2_6-15:18
- 挿入:317 [Insert]: Trunk_vertical_frame_04:1 ↔ M2_6-15:19
- 挿入:318 [Insert]: Trunk_vertical_frame_04:1 ↔ M2_6-15:20
- 挿入:319 [Insert]: Trunk_vertical_frame_04_MIR:1 ↔ M3-6:13
- 挿入:320 [Insert]: Trunk_vertical_frame_04_MIR:1 ↔ M3-6:14
- 挿入:321 [Insert]: Trunk_vertical_frame_04_MIR:1 ↔ M3-6:15
- 挿入:322 [Insert]: Trunk_vertical_frame_04_MIR:1 ↔ M3-6:16
- 挿入:323 [Insert]: Trunk_vertical_frame_04:1 ↔ M3-6:17
- 挿入:324 [Insert]: Trunk_vertical_frame_04:1 ↔ M3-6:18
- 挿入:325 [Insert]: Trunk_vertical_frame_04:1 ↔ M3-6:19
- 挿入:326 [Insert]: Trunk_vertical_frame_04:1 ↔ M3-6:20
- 挿入:327 [Insert]: Trunk_vertical_frame_03:1 ↔ M3-6:21
- 挿入:328 [Insert]: Trunk_vertical_frame_03:1 ↔ M3-6:22
- 挿入:329 [Insert]: Trunk_vertical_frame_03:1 ↔ M3-6:23
- 挿入:330 [Insert]: Trunk_vertical_frame_03:1 ↔ M3-6:24
- 挿入:331 [Insert]: Trunk_vertical_frame_03:2 ↔ M3-6:25
- 挿入:332 [Insert]: Trunk_vertical_frame_03:2 ↔ M3-6:26
- 挿入:333 [Insert]: Trunk_vertical_frame_03:2 ↔ M3-6:27
- 挿入:334 [Insert]: Trunk_vertical_frame_03:2 ↔ M3-6:28
- 挿入:335 [Insert]: Trunk_horizontal_frame_03:2 ↔ M2_6-20:9
- 挿入:336 [Insert]: Trunk_horizontal_frame_03:2 ↔ M2_6-20:10
- 挿入:337 [Insert]: Trunk_horizontal_frame_03:2 ↔ M2_6-20:11
- 挿入:338 [Insert]: Trunk_horizontal_frame_03:2 ↔ M2_6-20:12
- 挿入:339 [Insert]: Trunk_vertical_frame_06:2 ↔ M2_6-20:13
- 挿入:340 [Insert]: Trunk_vertical_frame_06:2 ↔ M2_6-20:16
- 挿入:341 [Insert]: Trunk_vertical_frame_06:2 ↔ M2_6-20:15
- 挿入:342 [Insert]: Trunk_vertical_frame_06:2 ↔ M2_6-20:14
- 挿入:343 [Insert]: Trunk_vertical_frame_06:1 ↔ M2_6-20:20
- 挿入:344 [Insert]: Trunk_vertical_frame_06:1 ↔ M2_6-20:17
- 挿入:345 [Insert]: Trunk_vertical_frame_06:1 ↔ M2_6-20:18
- 挿入:346 [Insert]: Trunk_vertical_frame_06:1 ↔ M2_6-20:19
- 挿入:347 [Insert]: Trunk_horizontal_frame_03:1 ↔ M3-6:29
- 挿入:348 [Insert]: Trunk_horizontal_frame_03:1 ↔ M3-6:30
- 挿入:349 [Insert]: Trunk_vertical_frame_03:1 ↔ M3-6:31
- 挿入:350 [Insert]: Trunk_vertical_frame_03:1 ↔ M3-6:32
- 挿入:351 [Insert]: Trunk_vertical_frame_03:2 ↔ M3-6:33
- 挿入:352 [Insert]: Trunk_vertical_frame_03:2 ↔ M3-6:34
- 挿入:371 [Insert]: Outer_support_stand:1 ↔ BRU-307S:1
- 挿入:372 [Insert]: Outer_support_stand:1 ↔ BRU-307S:2
- 挿入:373 [Insert]: Outer_support_stand:1 ↔ BRU-307S:3
- 挿入:374 [Insert]: Outer_support_stand:1 ↔ BRU-307S:4
- 挿入:375 [Insert]: Outer_support_stand:1 ↔ BRU-307S:5
- 挿入:376 [Insert]: Outer_support_stand:1 ↔ BRU-307S:6
- 挿入:377 [Insert]: Outer_support_stand:1 ↔ BRU-307S:7
- 挿入:378 [Insert]: Outer_support_stand:1 ↔ BRU-307S:8
- 挿入:391 [Insert]: B3M11xx:1 ↔ Inner_flange:1
- 挿入:392 [Insert]: B3M11xx:1 ↔ Inner_flange:1
- 挿入:397 [Insert]: Outer_support_stand:1 ↔ CRBA02508WWC8P5:1
- 角度:40 [Angle] (0 deg): Inner_support_stand:1 ↔ S3-07-3W:9
- 挿入:398 [Insert]: Inner_support_stand:1 ↔ S3-07-3W:9
- 角度:41 [Angle] (0 deg): Inner_support_stand:1 ↔ S3-07-3W:10
- 挿入:399 [Insert]: Inner_support_stand:1 ↔ S3-07-3W:10
- 角度:42 [Angle] (0 deg): Inner_support_stand:1 ↔ S3-07-3W:11
- 挿入:400 [Insert]: Inner_support_stand:1 ↔ S3-07-3W:11
- 角度:43 [Angle] (0 deg): Inner_support_stand:1 ↔ S3-07-3W:12
- 挿入:401 [Insert]: Inner_support_stand:1 ↔ S3-07-3W:12
- 挿入:404 [Insert]: BRU-307S:1 ↔ Outer_flange:1
- 挿入:405 [Insert]: BRU-307S:5 ↔ Outer_flange:1
- 挿入:406 [Insert]: Outer_flange:1 ↔ M3-6:35
- 挿入:407 [Insert]: Outer_flange:1 ↔ M3-6:36
- 挿入:408 [Insert]: Outer_flange:1 ↔ M3-6:37
- 挿入:409 [Insert]: Outer_flange:1 ↔ M3-6:38
- 挿入:410 [Insert]: Outer_flange:1 ↔ M3-6:39
- 挿入:411 [Insert]: Outer_flange:1 ↔ M3-6:40
- 挿入:412 [Insert]: Outer_flange:1 ↔ M3-6:41
- 挿入:413 [Insert]: Outer_flange:1 ↔ M3-6:42
- 挿入:418 [Insert]: Trunk_vertical_frame_01_MIR:1 ↔ Trunk_horizontal_frame_01:1
- 挿入:419 [Insert]: Trunk_vertical_frame_01_MIR:1 ↔ Trunk_horizontal_frame_01:1
- 挿入:420 [Insert]: Trunk_vertical_frame_01:1 ↔ Trunk_horizontal_frame_01:1
- 挿入:421 [Insert]: Trunk_vertical_frame_01:1 ↔ Trunk_horizontal_frame_01:1
- 挿入:422 [Insert]: B3M11xx:1 ↔ Trunk_horizontal_frame_01:1
- 挿入:423 [Insert]: B3M11xx:1 ↔ Trunk_horizontal_frame_01:1
- 挿入:424 [Insert]: B3M11xx:1 ↔ Trunk_horizontal_frame_01:1
- 挿入:425 [Insert]: B3M11xx:1 ↔ Trunk_horizontal_frame_01:1
- 挿入:426 [Insert]: Trunk_vertical_frame_01:1 ↔ Trunk_horizontal_frame_01:1
- 挿入:427 [Insert]: B3M11xx:2 ↔ Trunk_horizontal_frame_01:1
- 挿入:428 [Insert]: B3M11xx:2 ↔ Trunk_horizontal_frame_01:1
- 挿入:429 [Insert]: B3M11xx:2 ↔ Trunk_horizontal_frame_01:1
- 挿入:430 [Insert]: Trunk_horizontal_frame_01:1 ↔ SF319:1
- 挿入:431 [Insert]: Trunk_horizontal_frame_01:1 ↔ SF319:2
- 挿入:432 [Insert]: Trunk_horizontal_frame_01:1 ↔ SF319:3
- 挿入:433 [Insert]: Trunk_horizontal_frame_01:1 ↔ SF319:4
- 挿入:434 [Insert]: Trunk_horizontal_frame_01:1 ↔ SF319:5
- 挿入:435 [Insert]: Trunk_horizontal_frame_01:1 ↔ SF319:6
- 挿入:436 [Insert]: Trunk_horizontal_frame_01:1 ↔ SF319:7
- 挿入:438 [Insert]: Outer_support_stand:1 ↔ SF319:7
- 挿入:439 [Insert]: Outer_support_stand:1 ↔ SF319:4
- 挿入:440 [Insert]: Trunk_horizontal_frame_01:1 ↔ M2_6-15:22
- 挿入:441 [Insert]: Trunk_horizontal_frame_01:1 ↔ M2_6-15:21
- 挿入:442 [Insert]: Trunk_horizontal_frame_01:1 ↔ M2_6-15:23
- 挿入:443 [Insert]: Trunk_horizontal_frame_01:1 ↔ M2_6-15:24
- 挿入:444 [Insert]: Trunk_horizontal_frame_01:1 ↔ M2_6-15:25
- 挿入:445 [Insert]: Trunk_horizontal_frame_01:1 ↔ M2_6-15:26
- 挿入:446 [Insert]: Trunk_horizontal_frame_01:1 ↔ M2_6-15:27
- 挿入:447 [Insert]: Trunk_horizontal_frame_01:1 ↔ M2_6-15:28
- 挿入:448 [Insert]: Trunk_horizontal_frame_01:1 ↔ M3-8:13
- 挿入:449 [Insert]: Trunk_horizontal_frame_01:1 ↔ M3-8:14
- 挿入:450 [Insert]: Trunk_horizontal_frame_01:1 ↔ M3-8:15
- 挿入:451 [Insert]: Trunk_horizontal_frame_01:1 ↔ M3-8:16
- 挿入:452 [Insert]: Inner_flange:1 ↔ BRU-2609S:4
- 挿入:453 [Insert]: Inner_flange:1 ↔ BRU-2609S:3
- 挿入:454 [Insert]: Inner_flange:1 ↔ BRU-2609S:2
- 挿入:455 [Insert]: Inner_flange:1 ↔ BRU-2609S:1
- 挿入:456 [Insert]: Inner_support_stand:1 ↔ BRU-2609S:4
- 挿入:457 [Insert]: Inner_support_stand:1 ↔ BRU-2609S:1
- 挿入:458 [Insert]: Inner_support_stand:1 ↔ M2_6-8:1
- 挿入:459 [Insert]: Inner_support_stand:1 ↔ M2_6-8:2
- 挿入:460 [Insert]: Inner_support_stand:1 ↔ M2_6-8:3
- 挿入:461 [Insert]: Inner_support_stand:1 ↔ M2_6-8:4
- フラッシュ:22 [Flush]: Trunk_horizontal_frame_01:1
- 挿入:462 [Insert]: Trunk_horizontal_frame_01:1 ↔ SF319:8
